# Autodesk Inventor assembly: LED_module
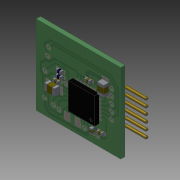
[picture p0: Inventor's stored thumbnail of the model, 180x180]
Saved by Autodesk Inventor 2013 (Build 170138000, 138)
## iProperties
Created: 2015-07-03
Part Number: LED_module
Document SubType Name: Assembly
Designer: terg
Author: terg
## Documents named in this file (11)
- C:\Users\terg\Projects\ModularElectronics\3D_models\LED_torch\LED_module.iam
- C:\Users\terg\Projects\ModularElectronics\3D_models\LED_torch\LED_module_PCB.ipt
- C:\Users\terg\Projects\ModularElectronics\3D_models\Components\0805_cap.ipt
- C:\Users\terg\Projects\ModularElectronics\3D_models\Components\0402_cap.ipt
- C:\Users\terg\Projects\ModularElectronics\3D_models\Components\0402_res.ipt
- C:\Users\terg\Projects\ModularElectronics\3D_models\Components\EFM32ZG110.ipt
- C:\Users\terg\Projects\ModularElectronics\3D_models\LED_torch\ADP1650.ipt
- C:\Users\terg\Projects\ModularElectronics\3D_models\LED_torch\XFL3010.ipt
- C:\Users\terg\Projects\ModularElectronics\3D_models\LED_torch\PowerLED.ipt
- C:\Users\terg\Projects\ModularElectronics\3D_models\Components\FemalConnector.ipt
- C:\Users\terg\Projects\ModularElectronics\3D_models\Components\MaleConnector.ipt
## Components (17 placed, 10 different names)
1. LED_module_PCB:1 — Zestawiający:1, Zestawiający:2, Równoległy:1, Równoległy:2, Równoległy:3, Równoległy:4, Zestawiający:3, Zestawiający:4, Równoległy:5, Równoległy:6, Równoległy:7, Równoległy:8, Zestawiający:5, Zestawiający:6, Zestawiający:7, Zestawiający:8, Równoległy:9, Równoległy:10, Równoległy:11, Równoległy:12, Równoległy:13, Równoległy:14, Równoległy:15, Równoległy:16, Zestawiający:9, Zestawiający:10, Równoległy:17, Równoległy:18, Równoległy:19, Równoległy:20, Zestawiający:11, Równoległy:21, Równoległy:22, Zestawiający:12, Równoległy:23, Równoległy:24, Zestawiający:13, Równoległy:25, Równoległy:26, Zestawiający:14, Zestawiający:15, Zestawiający:16, Równoległy:27, Równoległy:28, Równoległy:29, Równoległy:30
2. 0805_cap:1 — Zestawiający:1, Równoległy:1, Równoległy:2
3. 0805_cap:2 — Zestawiający:2, Równoległy:3, Równoległy:4
4. 0805_cap:3 — Zestawiający:3, Równoległy:5, Równoległy:8
5. 0805_cap:4 — Zestawiający:4, Równoległy:6, Równoległy:7
6. 0402_cap:1 — Zestawiający:5, Równoległy:13, Równoległy:14
7. 0402_cap:2 — Zestawiający:6, Równoległy:15, Równoległy:16
8. 0402_cap:3 — Zestawiający:8, Równoległy:9, Równoległy:10
9. 0402_cap:4 — Zestawiający:7, Równoległy:11, Równoległy:12
10. 0402_res:1 — Zestawiający:9, Równoległy:17, Równoległy:20
11. 0402_res:2 — Zestawiający:10, Równoległy:18, Równoległy:19
12. EFM32ZG110:1 — Zestawiający:11, Równoległy:21, Równoległy:22
13. ADP1650:1 — Zestawiający:12, Równoległy:23, Równoległy:24
14. XFL3010:1 — Zestawiający:13, Równoległy:25, Równoległy:26
15. PowerLED:1 — Zestawiający:14
16. FemalConnector:1 — Zestawiający:15, Równoległy:27, Równoległy:28
17. MaleConnector:1 — Zestawiający:16, Równoległy:29, Równoległy:30
## Relationships (46: Flush 30, Mate 16)
- Zestawiający:1 [Mate]: LED_module_PCB:1 ↔ 0805_cap:1
- Zestawiający:2 [Mate]: LED_module_PCB:1 ↔ 0805_cap:2
- Równoległy:1 [Flush] (0.928 mm): LED_module_PCB:1 ↔ 0805_cap:1
- Równoległy:2 [Flush] (1.318 mm): LED_module_PCB:1 ↔ 0805_cap:1
- Równoległy:3 [Flush] (5.432 mm): LED_module_PCB:1 ↔ 0805_cap:2
- Równoległy:4 [Flush] (11.435 mm): LED_module_PCB:1 ↔ 0805_cap:2
- Zestawiający:3 [Mate]: LED_module_PCB:1 ↔ 0805_cap:3
- Zestawiający:4 [Mate]: LED_module_PCB:1 ↔ 0805_cap:4
- Równoległy:5 [Flush] (11.525 mm): LED_module_PCB:1 ↔ 0805_cap:3
- Równoległy:6 [Flush] (2.248 mm): LED_module_PCB:1 ↔ 0805_cap:4
- Równoległy:7 [Flush] (9.42 mm): LED_module_PCB:1 ↔ 0805_cap:4
- Równoległy:8 [Flush] (4.958 mm): LED_module_PCB:1 ↔ 0805_cap:3
- Zestawiający:5 [Mate]: LED_module_PCB:1 ↔ 0402_cap:1
- Zestawiający:6 [Mate]: LED_module_PCB:1 ↔ 0402_cap:2
- Zestawiający:7 [Mate]: LED_module_PCB:1 ↔ 0402_cap:4
- Zestawiający:8 [Mate]: LED_module_PCB:1 ↔ 0402_cap:3
- Równoległy:9 [Flush] (1.684 mm): LED_module_PCB:1 ↔ 0402_cap:3
- Równoległy:10 [Flush] (4.971 mm): LED_module_PCB:1 ↔ 0402_cap:3
- Równoległy:11 [Flush] (3.105 mm): LED_module_PCB:1 ↔ 0402_cap:4
- Równoległy:12 [Flush] (2.379 mm): LED_module_PCB:1 ↔ 0402_cap:4
- Równoległy:13 [Flush] (6.696 mm): LED_module_PCB:1 ↔ 0402_cap:1
- Równoległy:14 [Flush] (11.397 mm): LED_module_PCB:1 ↔ 0402_cap:1
- Równoległy:15 [Flush] (5.412 mm): LED_module_PCB:1 ↔ 0402_cap:2
- Równoległy:16 [Flush] (9.795 mm): LED_module_PCB:1 ↔ 0402_cap:2
- Zestawiający:9 [Mate]: LED_module_PCB:1 ↔ 0402_res:1
- Zestawiający:10 [Mate]: LED_module_PCB:1 ↔ 0402_res:2
- Równoległy:17 [Flush] (4.145 mm): LED_module_PCB:1 ↔ 0402_res:1
- Równoległy:18 [Flush] (4.173 mm): LED_module_PCB:1 ↔ 0402_res:2
- Równoległy:19 [Flush] (5.871 mm): LED_module_PCB:1 ↔ 0402_res:2
- Równoległy:20 [Flush] (6.758 mm): LED_module_PCB:1 ↔ 0402_res:1
- Zestawiający:11 [Mate]: LED_module_PCB:1 ↔ EFM32ZG110:1
- Równoległy:21 [Flush] (4.086 mm): LED_module_PCB:1 ↔ EFM32ZG110:1
- Równoległy:22 [Flush] (3.741 mm): LED_module_PCB:1 ↔ EFM32ZG110:1
- Zestawiający:12 [Mate]: LED_module_PCB:1 ↔ ADP1650:1
- Równoległy:23 [Flush] (1.6 mm): LED_module_PCB:1 ↔ ADP1650:1
- Równoległy:24 [Flush] (7.306 mm): LED_module_PCB:1 ↔ ADP1650:1
- Zestawiający:13 [Mate]: LED_module_PCB:1 ↔ XFL3010:1
- Równoległy:25 [Flush] (1.176 mm): LED_module_PCB:1 ↔ XFL3010:1
- Równoległy:26 [Flush] (10.167 mm): LED_module_PCB:1 ↔ XFL3010:1
- Zestawiający:14 [Mate]: LED_module_PCB:1 ↔ PowerLED:1
- Zestawiający:15 [Mate]: LED_module_PCB:1 ↔ FemalConnector:1
- Zestawiający:16 [Mate]: LED_module_PCB:1 ↔ MaleConnector:1
- Równoległy:27 [Flush] (3.511 mm): LED_module_PCB:1 ↔ FemalConnector:1
- Równoległy:28 [Flush] (-0.816 mm): LED_module_PCB:1 ↔ FemalConnector:1
- Równoległy:29 [Flush] (4.053 mm): LED_module_PCB:1 ↔ MaleConnector:1
- Równoległy:30 [Flush] (3.343 mm): LED_module_PCB:1 ↔ MaleConnector:1
